# Autodesk Inventor assembly: złożenie2
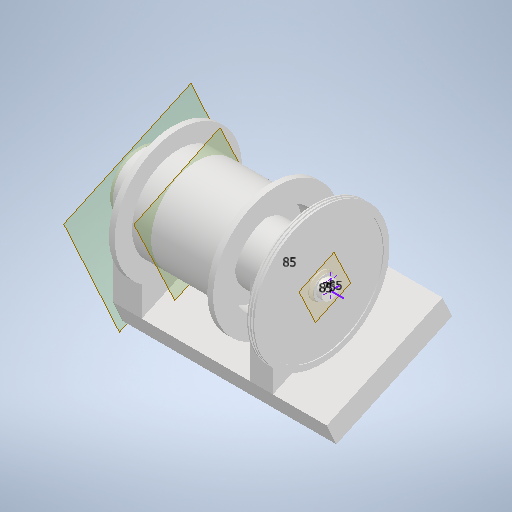
[picture p0: Inventor's stored thumbnail of the model, 512x512]
Saved by Autodesk Inventor 2025 (Build 290162000, 162)
## iProperties
Created: 2025-05-18
Part Number: złożenie2
Document SubType Name: Assembly
Designer: PC
Author: PC
## Documents named in this file (14)
- C:\Users\failc\Desktop\pkmpkm\src\Assemblies\złożenie2.iam
- C:\Users\failc\Desktop\pkmpkm\src\Parts\Wał4.ipt
- C:\Users\failc\Desktop\pkmpkm\src\Parts\1415151513515.ipt
- C:\Users\failc\Desktop\pkmpkm\src\ContentCenter\pl-PL\BS 290 SKF(05)\BS 290 SKF - SKF QJ 230 N2.ipt
- C:\Users\failc\Desktop\pkmpkm\src\Assemblies\Połączenie wpustowe1.iam
- C:\Users\failc\Desktop\pkmpkm\src\Assemblies\Połączenie wpustowe2.iam
- C:\Users\failc\Desktop\pkmpkm\src\Parts\podstawa.ipt
- C:\Users\failc\Desktop\pkmpkm\src\ContentCenter\pl-PL\DIN 705   B\DIN 705 - B150.ipt
- C:\Users\failc\Desktop\pkmpkm\pięćśetka.ipt
- C:\Users\failc\Desktop\pkmpkm\src\ContentCenter\pl-PL\AS 1110\AS 1110 - M36 x 60.ipt
- C:\Users\failc\Desktop\pkmpkm\src\ContentCenter\pl-PL\DIN 3760 A\DIN 3760 - A - 150 x 180 x 15 - NBR.ipt
- C:\Users\failc\Desktop\pkmpkm\src\Assemblies\złożenie2\Design Accelerator\Połączenie wpustowe1.iam
- C:\Users\failc\Downloads\koło zębate2 (1).ipt
- C:\Users\failc\Desktop\pkmpkm\src\Assemblies\złożenie2\Design Accelerator\Połączenie wpustowe2.iam
## Components (23 placed, 10 different names)
1. Wał:1 — Równoległe:1, Zestawiające:4, Kątowe:3, Kątowe:5, Równoległe:5, Kątowe:7, Zestawiające:7, Równoległe:6, Kątowe:8, Zestawiające:8, Kątowe:9, Zestawiające:9, Równoległe:7, Równoległe:8, Kątowe:10, Zestawiające:10
2. 1415151513515:1 — Zestawiające:4, Kątowe:3, Kątowe:5, Kątowe:9
3. BS 290 SKF- do styku czteropunktowego SKF QJ 230 N2:1 — Obrotowe:1
4. BS 290 SKF- do styku czteropunktowego SKF QJ 230 N2:2 — Walcowe:1, Obrotowe:2
5. Połączenie wpustowe:1 [sub-assembly] — Równoległe:5, Kątowe:7, Zestawiające:7
6. Połączenie wpustowe:2 [sub-assembly] — Równoległe:6, Kątowe:8, Zestawiające:8
7. podstawa:1 — Walcowe:1, Obrotowe:3, Obrotowe:4, Obrotowe:5, Obrotowe:6, Obrotowe:7, Obrotowe:8, Obrotowe:9, Obrotowe:10, Obrotowe:12
8. DIN 705 B B150:1 — Obrotowe:1
9. DIN 705 B B150:2 — Obrotowe:2
10. pięćśetka:1 — Obrotowe:3
11. AS 1110 - Metryczny M36 x 60:1 — Obrotowe:7
12. AS 1110 - Metryczny M36 x 60:2 — Obrotowe:5
13. AS 1110 - Metryczny M36 x 60:3 — Obrotowe:6
14. AS 1110 - Metryczny M36 x 60:4 — Obrotowe:4
15. DIN 3760 A A - 150 x 180 x 15 - NBR:1 — Sztywne:1
16. pięćśetka:2 — Obrotowe:8, Sztywne:1, Obrotowe:11
17. AS 1110 - Metryczny M36 x 60:5 — Obrotowe:10
18. AS 1110 - Metryczny M36 x 60:6 — Obrotowe:9
19. AS 1110 - Metryczny M36 x 60:7 — Obrotowe:11
20. AS 1110 - Metryczny M36 x 60:8 — Obrotowe:12
21. koło zębate2 (1):1 — Zestawiające:9
22. Połączenie wpustowe:3 [sub-assembly] — Równoległe:8, Kątowe:10, Zestawiające:10
23. Połączenie wpustowe:4 [sub-assembly]
## Relationships (31: RevoluteJoint 12, Flush 6, Angle 6, Mate 5, CylindricalJoint 1, WeldJoint 1)
- Równoległe:1 [Flush]: Wał:1
- Równoległe:2 [Flush] (-200 mm)
- Zestawiające:4 [Mate] (180 mm): Wał:1 ↔ 1415151513515:1
- Kątowe:3 [Angle] (90 deg): Wał:1 ↔ 1415151513515:1
- Kątowe:5 [Angle] (90 deg): Wał:1 ↔ 1415151513515:1
- Równoległe:5 [Flush] (204.9231 mm): Wał:1 ↔ Połączenie wpustowe:1
- Kątowe:7 [Angle] (180 deg): Wał:1 ↔ Połączenie wpustowe:1
- Zestawiające:7 [Mate]: Wał:1 ↔ Połączenie wpustowe:1
- Równoległe:6 [Flush] (204.9722 mm): Wał:1 ↔ Połączenie wpustowe:2
- Kątowe:8 [Angle] (0 deg): Wał:1 ↔ Połączenie wpustowe:2
- Zestawiające:8 [Mate]: Wał:1 ↔ Połączenie wpustowe:2
- Kątowe:9 [Angle] (90 deg): Wał:1 ↔ 1415151513515:1
- Walcowe:1 [CylindricalJoint]: BS 290 SKF- do styku czteropunktowego SKF QJ 230 N2:2 ↔ podstawa:1
- Obrotowe:1 [RevoluteJoint]: BS 290 SKF- do styku czteropunktowego SKF QJ 230 N2:1 ↔ DIN 705 B B150:1
- Obrotowe:2 [RevoluteJoint]: BS 290 SKF- do styku czteropunktowego SKF QJ 230 N2:2 ↔ DIN 705 B B150:2
- Obrotowe:3 [RevoluteJoint]: podstawa:1 ↔ pięćśetka:1
- Obrotowe:4 [RevoluteJoint]: podstawa:1 ↔ AS 1110 - Metryczny M36 x 60:4
- Obrotowe:5 [RevoluteJoint]: podstawa:1 ↔ AS 1110 - Metryczny M36 x 60:2
- Obrotowe:6 [RevoluteJoint]: podstawa:1 ↔ AS 1110 - Metryczny M36 x 60:3
- Obrotowe:7 [RevoluteJoint]: podstawa:1 ↔ AS 1110 - Metryczny M36 x 60:1
- Obrotowe:8 [RevoluteJoint]: podstawa:1 ↔ pięćśetka:2
- Sztywne:1 [WeldJoint] (10 mm): DIN 3760 A A - 150 x 180 x 15 - NBR:1 ↔ pięćśetka:2
- Obrotowe:9 [RevoluteJoint] (-35 mm): podstawa:1 ↔ AS 1110 - Metryczny M36 x 60:6
- Obrotowe:10 [RevoluteJoint] (35 mm): podstawa:1 ↔ AS 1110 - Metryczny M36 x 60:5
- Obrotowe:11 [RevoluteJoint] (-35 mm): pięćśetka:2 ↔ AS 1110 - Metryczny M36 x 60:7
- Obrotowe:12 [RevoluteJoint]: podstawa:1 ↔ AS 1110 - Metryczny M36 x 60:8
- Zestawiające:9 [Mate] (47 mm): Wał:1 ↔ koło zębate2 (1):1
- Równoległe:7 [Flush] (-50 mm): Wał:1
- Równoległe:8 [Flush] (56.6721 mm): Wał:1 ↔ Połączenie wpustowe:3
- Kątowe:10 [Angle] (180 deg): Wał:1 ↔ Połączenie wpustowe:3
- Zestawiające:10 [Mate]: Wał:1 ↔ Połączenie wpustowe:3
